# Autodesk Inventor assembly: ASY PNS 750 filter-distribution-system 1200
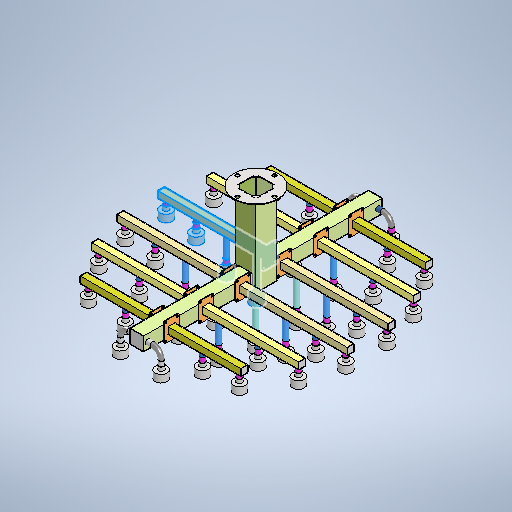
[picture p0: Inventor's stored thumbnail of the model, 512x512]
Saved by Autodesk Inventor 2025.1 (Build 291241020, 241B)
## iProperties
Created: 2025-06-24
Part Number: ASY PNS 750 filter-distribution-system 1200
Document SubType Name: Assembly
Designer: user
Author: user
## Documents named in this file (14)
- C:\Users\user\YandexDisk-badmisterfox\home pc\Inventor\PNS2-Panaevsk\filter-distribution-system\ASY PNS 750 filter-distribution-system 1200.iam
- C:\Users\user\YandexDisk-badmisterfox\home pc\Inventor\PNS2-Panaevsk\filter-distribution-system\PNS 751 DIM filter-distribution-system 1200.ipt
- C:\Users\user\YandexDisk-badmisterfox\home pc\Inventor\PNS2-Panaevsk\filter-distribution-system\PNS 754 FDS 1200 FLANGE.ipt
- C:\Users\user\YandexDisk-badmisterfox\home pc\Inventor\PNS2-Panaevsk\filter-distribution-system\PNS 752 FDS 1200 FLANGE 2.ipt
- C:\Users\user\YandexDisk-badmisterfox\home pc\Inventor\PNS2-Panaevsk\filter-distribution-system\PNS 753 FDS 1200 FLANGE 3.ipt
- C:\Users\user\YandexDisk-badmisterfox\home pc\Inventor\PNS2-Panaevsk\CC\en-US\JIS B 2312 90 (4)\JIS B 2312 90 Deg Long Elbow Stainless Steel 15A x Sch 5S.ipt
- C:\Users\user\YandexDisk-badmisterfox\home pc\Inventor\PNS2-Panaevsk\PNS dummy filter element.ipt
- C:\Users\user\YandexDisk-badmisterfox\home pc\Inventor\PNS2-Panaevsk\PNS dummy pipe nippel.ipt
- C:\Users\user\YandexDisk-badmisterfox\home pc\Inventor\PNS2-Panaevsk\filter-distribution-system\PNS 759 FDS 1200 way tube 7.ipt
- C:\Users\user\YandexDisk-badmisterfox\home pc\Inventor\PNS2-Panaevsk\filter-distribution-system\ASY PNS FDS way1.iam
- C:\Users\user\YandexDisk-badmisterfox\home pc\Inventor\PNS2-Panaevsk\filter-distribution-system\ASY PNS FDS way 2.iam
- C:\Users\user\YandexDisk-badmisterfox\home pc\Inventor\PNS2-Panaevsk\filter-distribution-system\ASY PNS FDS way3.iam
- C:\Users\user\YandexDisk-badmisterfox\home pc\Inventor\PNS2-Panaevsk\filter-distribution-system\PNS 767 FDS 1200 CUP 2.ipt
- C:\Users\user\YandexDisk-badmisterfox\home pc\Inventor\PNS2-Panaevsk\filter-distribution-system\PNS 765 FDS 1200 CUP 1.ipt
## Components (37 placed, 14 different names)
1. Dimensions:1 — Mate:4, Mate:5
2. PNS FDS 1200 FLANGE:1 — Mate:1, Flush:1, Flush:2
3. PNS FDS 1200 FLANGE 2:1 — Rigid:1, Flush:1, Rigid:2, Mate:6, Flush:3, Flush:4
4. PNS FDS 1200 FLANGE 2:2 — Rigid:1, Mate:1, Flush:2, Rigid:3
5. PNS FDS 1200 FLANGE 3:1 — Rigid:2, Rigid:7, Rigid:9, Rigid:14, Rigid:15, Rigid:31, Rigid:33
6. PNS 753 FDS 1200 FLANGE 3:2 — Rigid:3, Rigid:10, Rigid:11, Rigid:12, Rigid:13, Rigid:16, Rigid:17, Rigid:29, Rigid:30, Rigid:32
7. JIS B 2312 90 Deg Long Elbow Stainless Steel 15A x Sch 5S:1 — Rigid:7, Rigid:8, Rigid:18, Rigid:19
8. PNS dummy filter element:1 — Rigid:8
9. PNS dummy pipe nippel:1 — Rigid:18
10. ASY PNS FDS way1:1 [sub-assembly]
11. ASY PNS FDS way 2:1 [sub-assembly]
12. ASY PNS FDS way3:1 [sub-assembly]
13. ASY PNS FDS way1:2 [sub-assembly] — Rigid:9
14. ASY PNS FDS way1:3 [sub-assembly] — Rigid:11
15. ASY PNS FDS way1:4 [sub-assembly] — Rigid:10
16. ASY PNS FDS way 2:2 [sub-assembly] — Rigid:14
17. ASY PNS FDS way 2:3 [sub-assembly] — Rigid:13
18. ASY PNS FDS way 2:4 [sub-assembly] — Rigid:12
19. ASY PNS FDS way3:2 [sub-assembly] — Rigid:15
20. ASY PNS FDS way3:3 [sub-assembly] — Rigid:16
21. ASY PNS FDS way3:4 [sub-assembly] — Rigid:17
22. PNS 759 FDS 1200 way tube 7:1 — Rigid:19
23. JIS B 2312 90 Deg Long Elbow Stainless Steel 15A x Sch 5S:2
24. PNS dummy filter element:2
25. PNS dummy pipe nippel:2
26. PNS 759 FDS 1200 way tube 7:2 — Rigid:31
27. JIS B 2312 90 Deg Long Elbow Stainless Steel 15A x Sch 5S:3
28. PNS dummy filter element:3
29. PNS dummy pipe nippel:3
30. PNS 759 FDS 1200 way tube 7:3 — Rigid:29
31. JIS B 2312 90 Deg Long Elbow Stainless Steel 15A x Sch 5S:4
32. PNS dummy filter element:4
33. PNS dummy pipe nippel:4
34. PNS 759 FDS 1200 way tube 7:4 — Rigid:30
35. PNS 767 FDS 1200 CUP 2:1 — Rigid:32
36. PNS 767 FDS 1200 CUP 2:2 — Rigid:33
37. PNS 765 FDS 1200 CUP 1:1 — Mate:6, Flush:3, Flush:4
## Relationships (41: WeldJoint 33, Mate 4, Flush 4)
- Rigid:1 [WeldJoint]: PNS FDS 1200 FLANGE 2:1 ↔ PNS FDS 1200 FLANGE 2:2
- Mate:1: PNS FDS 1200 FLANGE:1 ↔ PNS FDS 1200 FLANGE 2:2
- Flush:1: PNS FDS 1200 FLANGE:1 ↔ PNS FDS 1200 FLANGE 2:1
- Flush:2: PNS FDS 1200 FLANGE:1 ↔ PNS FDS 1200 FLANGE 2:2
- Mate:4: Dimensions:1
- Mate:5: Dimensions:1
- Rigid:2 [WeldJoint]: PNS FDS 1200 FLANGE 2:1 ↔ PNS FDS 1200 FLANGE 3:1
- Rigid:3 [WeldJoint]: PNS FDS 1200 FLANGE 2:2 ↔ PNS 753 FDS 1200 FLANGE 3:2
- [WeldJoint] (-2 mm): PNS FDS 1200 FLANGE 3:1 ↔ ASY PNS FDS way1:1
- [WeldJoint] (-2 mm): PNS FDS 1200 FLANGE 3:1 ↔ ASY PNS FDS way 2:1
- [WeldJoint]: PNS FDS 1200 FLANGE 3:1 ↔ ASY PNS FDS way3:1
- Rigid:7 [WeldJoint] (-20 mm): PNS FDS 1200 FLANGE 3:1 ↔ JIS B 2312 90 Deg Long Elbow Stainless Steel 15A x Sch 5S:1
- Rigid:8 [WeldJoint] (20 mm): JIS B 2312 90 Deg Long Elbow Stainless Steel 15A x Sch 5S:1 ↔ PNS dummy filter element:1
- Rigid:9 [WeldJoint]: PNS FDS 1200 FLANGE 3:1 ↔ ASY PNS FDS way1:2
- Rigid:10 [WeldJoint]: PNS 753 FDS 1200 FLANGE 3:2 ↔ ASY PNS FDS way1:4
- Rigid:11 [WeldJoint]: PNS 753 FDS 1200 FLANGE 3:2 ↔ ASY PNS FDS way1:3
- Rigid:12 [WeldJoint]: PNS 753 FDS 1200 FLANGE 3:2 ↔ ASY PNS FDS way 2:4
- Rigid:13 [WeldJoint]: PNS 753 FDS 1200 FLANGE 3:2 ↔ ASY PNS FDS way 2:3
- Rigid:14 [WeldJoint]: PNS FDS 1200 FLANGE 3:1 ↔ ASY PNS FDS way 2:2
- Rigid:15 [WeldJoint]: PNS FDS 1200 FLANGE 3:1 ↔ ASY PNS FDS way3:2
- Rigid:16 [WeldJoint]: PNS 753 FDS 1200 FLANGE 3:2 ↔ ASY PNS FDS way3:3
- Rigid:17 [WeldJoint]: PNS 753 FDS 1200 FLANGE 3:2 ↔ ASY PNS FDS way3:4
- Rigid:18 [WeldJoint]: JIS B 2312 90 Deg Long Elbow Stainless Steel 15A x Sch 5S:1 ↔ PNS dummy pipe nippel:1
- Rigid:19 [WeldJoint]: JIS B 2312 90 Deg Long Elbow Stainless Steel 15A x Sch 5S:1 ↔ PNS 759 FDS 1200 way tube 7:1
- [WeldJoint] (20 mm): JIS B 2312 90 Deg Long Elbow Stainless Steel 15A x Sch 5S:2 ↔ PNS dummy filter element:2
- [WeldJoint]: JIS B 2312 90 Deg Long Elbow Stainless Steel 15A x Sch 5S:2 ↔ PNS dummy pipe nippel:2
- [WeldJoint]: JIS B 2312 90 Deg Long Elbow Stainless Steel 15A x Sch 5S:2 ↔ PNS 759 FDS 1200 way tube 7:2
- [WeldJoint] (20 mm): JIS B 2312 90 Deg Long Elbow Stainless Steel 15A x Sch 5S:3 ↔ PNS dummy filter element:3
- [WeldJoint]: JIS B 2312 90 Deg Long Elbow Stainless Steel 15A x Sch 5S:3 ↔ PNS dummy pipe nippel:3
- [WeldJoint]: JIS B 2312 90 Deg Long Elbow Stainless Steel 15A x Sch 5S:3 ↔ PNS 759 FDS 1200 way tube 7:3
- [WeldJoint] (20 mm): JIS B 2312 90 Deg Long Elbow Stainless Steel 15A x Sch 5S:4 ↔ PNS dummy filter element:4
- [WeldJoint]: JIS B 2312 90 Deg Long Elbow Stainless Steel 15A x Sch 5S:4 ↔ PNS dummy pipe nippel:4
- [WeldJoint]: JIS B 2312 90 Deg Long Elbow Stainless Steel 15A x Sch 5S:4 ↔ PNS 759 FDS 1200 way tube 7:4
- Rigid:29 [WeldJoint]: PNS 753 FDS 1200 FLANGE 3:2 ↔ PNS 759 FDS 1200 way tube 7:3
- Rigid:30 [WeldJoint]: PNS 753 FDS 1200 FLANGE 3:2 ↔ PNS 759 FDS 1200 way tube 7:4
- Rigid:31 [WeldJoint]: PNS FDS 1200 FLANGE 3:1 ↔ PNS 759 FDS 1200 way tube 7:2
- Rigid:32 [WeldJoint]: PNS 753 FDS 1200 FLANGE 3:2 ↔ PNS 767 FDS 1200 CUP 2:1
- Rigid:33 [WeldJoint]: PNS FDS 1200 FLANGE 3:1 ↔ PNS 767 FDS 1200 CUP 2:2
- Mate:6: PNS FDS 1200 FLANGE 2:1 ↔ PNS 765 FDS 1200 CUP 1:1
- Flush:3: PNS FDS 1200 FLANGE 2:1 ↔ PNS 765 FDS 1200 CUP 1:1
- Flush:4: PNS FDS 1200 FLANGE 2:1 ↔ PNS 765 FDS 1200 CUP 1:1
## Named parameters: d69_d30 = 20 mm, d70_d67 = 0 mm, d71_d68 = 0 mm, d72_d30 = 20 mm, d73_d67 = 0 mm, d74_d68 = 0 mm, d75_d30 = 20 mm, d76_d67 = 0 mm, d77_d68 = 0 mm
